# Autodesk Inventor assembly: vrRig_v01r1_bpBox
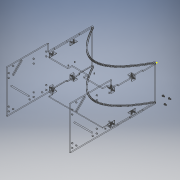
[picture p0: Inventor's stored thumbnail of the model, 180x180]
Saved by Autodesk Inventor 2016 (Build 200138000, 138)
## iProperties
Created: 2019-01-03
Part Number: vrRig_v01r1_bpBox
Document SubType Name: Assembly
Designer: harveylab
Author: harveylab
## Documents named in this file (6)
- C:\Users\harveylab\Documents\GitHub\HarVR\Hardware\BackProjection\vrRig_v01r1_bpBox.iam
- C:\Users\harveylab\Documents\GitHub\HarVR\Hardware\BackProjection\vrRig_v01r1_bottom.ipt
- C:\Users\harveylab\Documents\GitHub\HarVR\Hardware\BackProjection\McM_47065T236_cornerBracket_1in.ipt
- C:\Users\harveylab\Documents\GitHub\HarVR\Hardware\BackProjection\McM_92220A182_lowProfScrew_0p375in.ipt
- C:\Users\harveylab\Documents\GitHub\HarVR\Hardware\BackProjection\vrRig_v01r1_side.ipt
- C:\Users\harveylab\Documents\GitHub\HarVR\Hardware\BackProjection\vrRig_v01r1_top.ipt
## Components (28 placed, 5 different names)
1. vrRig_v01r1_bottom:1 — Mate:1, Insert:1, Insert:2, Insert:3, Insert:4, Flush:1, Flush:2, Flush:3, Flush:4
2. McM_47065T236_cornerBracket_1in:1 — Insert:1, Flush:4, Insert:7, Insert:9, Insert:15
3. McM_47065T236_cornerBracket_1in:2 — Insert:2, Flush:3, Insert:8, Insert:10, Insert:16
4. McM_47065T236_cornerBracket_1in:3 — Insert:4, Flush:1, Insert:6, Insert:11, Insert:14
5. McM_47065T236_cornerBracket_1in:4 — Insert:3, Flush:2, Insert:5, Insert:12, Insert:13
6. McM_92220A182_lowProfScrew_0p375in:1 — Insert:5
7. McM_92220A182_lowProfScrew_0p375in:2 — Insert:6
8. McM_92220A182_lowProfScrew_0p375in:3 — Insert:8
9. McM_92220A182_lowProfScrew_0p375in:4 — Insert:7
10. vrRig_v01r1_side:1 — Insert:9, Insert:10, Insert:17, Insert:18, Flush:5, Flush:6
11. vrRig_v01r1_side:2 — Insert:11, Insert:12, Insert:19, Insert:20, Flush:7, Flush:8
12. McM_92220A182_lowProfScrew_0p375in:5 — Insert:14
13. McM_92220A182_lowProfScrew_0p375in:6 — Insert:13
14. McM_92220A182_lowProfScrew_0p375in:7 — Insert:16
15. McM_92220A182_lowProfScrew_0p375in:8 — Insert:15
16. McM_47065T236_cornerBracket_1in:5 — Insert:20, Flush:8
17. McM_47065T236_cornerBracket_1in:6 — Insert:18, Flush:5, Insert:21, Insert:25, Insert:26
18. McM_47065T236_cornerBracket_1in:7 — Insert:17, Flush:6, Insert:23, Insert:24
19. McM_47065T236_cornerBracket_1in:8 — Insert:19, Flush:7, Insert:22, Insert:27
20. vrRig_v01r1_top:1 — Insert:21, Insert:22
21. McM_92220A182_lowProfScrew_0p375in:9 — Insert:24
22. McM_92220A182_lowProfScrew_0p375in:10 — Insert:26
23. McM_92220A182_lowProfScrew_0p375in:11
24. McM_92220A182_lowProfScrew_0p375in:12
25. McM_92220A182_lowProfScrew_0p375in:13
26. McM_92220A182_lowProfScrew_0p375in:14 — Insert:27
27. McM_92220A182_lowProfScrew_0p375in:15 — Insert:25
28. McM_92220A182_lowProfScrew_0p375in:16 — Insert:23
## Relationships (36: Insert 27, Flush 8, Mate 1)
- Mate:1: vrRig_v01r1_bottom:1
- Insert:1: vrRig_v01r1_bottom:1 ↔ McM_47065T236_cornerBracket_1in:1
- Insert:2: vrRig_v01r1_bottom:1 ↔ McM_47065T236_cornerBracket_1in:2
- Insert:3: vrRig_v01r1_bottom:1 ↔ McM_47065T236_cornerBracket_1in:4
- Insert:4: vrRig_v01r1_bottom:1 ↔ McM_47065T236_cornerBracket_1in:3
- Flush:1: vrRig_v01r1_bottom:1 ↔ McM_47065T236_cornerBracket_1in:3
- Flush:2: vrRig_v01r1_bottom:1 ↔ McM_47065T236_cornerBracket_1in:4
- Flush:3: vrRig_v01r1_bottom:1 ↔ McM_47065T236_cornerBracket_1in:2
- Flush:4: vrRig_v01r1_bottom:1 ↔ McM_47065T236_cornerBracket_1in:1
- Insert:5 (-9.525 mm): McM_47065T236_cornerBracket_1in:4 ↔ McM_92220A182_lowProfScrew_0p375in:1
- Insert:6: McM_47065T236_cornerBracket_1in:3 ↔ McM_92220A182_lowProfScrew_0p375in:2
- Insert:7: McM_47065T236_cornerBracket_1in:1 ↔ McM_92220A182_lowProfScrew_0p375in:4
- Insert:8: McM_47065T236_cornerBracket_1in:2 ↔ McM_92220A182_lowProfScrew_0p375in:3
- Insert:9: McM_47065T236_cornerBracket_1in:1 ↔ vrRig_v01r1_side:1
- Insert:10: McM_47065T236_cornerBracket_1in:2 ↔ vrRig_v01r1_side:1
- Insert:11: McM_47065T236_cornerBracket_1in:3 ↔ vrRig_v01r1_side:2
- Insert:12: McM_47065T236_cornerBracket_1in:4 ↔ vrRig_v01r1_side:2
- Insert:13: McM_47065T236_cornerBracket_1in:4 ↔ McM_92220A182_lowProfScrew_0p375in:6
- Insert:14: McM_47065T236_cornerBracket_1in:3 ↔ McM_92220A182_lowProfScrew_0p375in:5
- Insert:15: McM_47065T236_cornerBracket_1in:1 ↔ McM_92220A182_lowProfScrew_0p375in:8
- Insert:16: McM_47065T236_cornerBracket_1in:2 ↔ McM_92220A182_lowProfScrew_0p375in:7
- Insert:17: vrRig_v01r1_side:1 ↔ McM_47065T236_cornerBracket_1in:7
- Insert:18: vrRig_v01r1_side:1 ↔ McM_47065T236_cornerBracket_1in:6
- Insert:19: vrRig_v01r1_side:2 ↔ McM_47065T236_cornerBracket_1in:8
- Insert:20: vrRig_v01r1_side:2 ↔ McM_47065T236_cornerBracket_1in:5
- Flush:5: vrRig_v01r1_side:1 ↔ McM_47065T236_cornerBracket_1in:6
- Flush:6: vrRig_v01r1_side:1 ↔ McM_47065T236_cornerBracket_1in:7
- Flush:7: vrRig_v01r1_side:2 ↔ McM_47065T236_cornerBracket_1in:8
- Flush:8: vrRig_v01r1_side:2 ↔ McM_47065T236_cornerBracket_1in:5
- Insert:21: McM_47065T236_cornerBracket_1in:6 ↔ vrRig_v01r1_top:1
- Insert:22: McM_47065T236_cornerBracket_1in:8 ↔ vrRig_v01r1_top:1
- Insert:23: McM_47065T236_cornerBracket_1in:7 ↔ McM_92220A182_lowProfScrew_0p375in:16
- Insert:24: McM_47065T236_cornerBracket_1in:7 ↔ McM_92220A182_lowProfScrew_0p375in:9
- Insert:25: McM_47065T236_cornerBracket_1in:6 ↔ McM_92220A182_lowProfScrew_0p375in:15
- Insert:26: McM_47065T236_cornerBracket_1in:6 ↔ McM_92220A182_lowProfScrew_0p375in:10
- Insert:27: McM_47065T236_cornerBracket_1in:8 ↔ McM_92220A182_lowProfScrew_0p375in:14
